# Autodesk Inventor assembly: 13
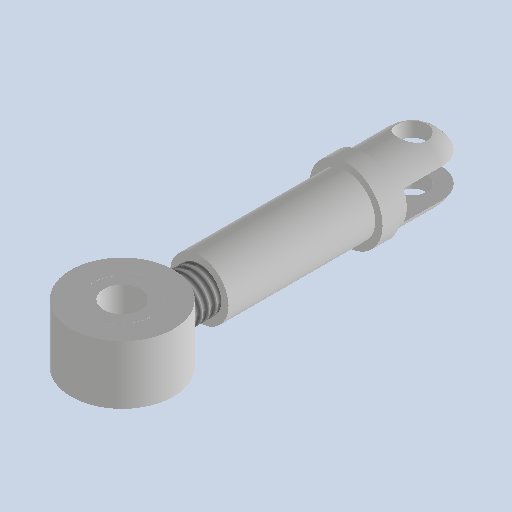
[picture p0: Inventor's stored thumbnail of the model, 512x512]
Saved by Autodesk Inventor 2025.1 (Build 291241000, 241)
## iProperties
Created: 2024-09-13
Part Number: 13
Document SubType Name: Assembly
Designer: ffogue
Author: ffogue
## Documents named in this file (4)
- C:\Users\ffogue\Documents\Inventor\Single cylinder Steam Engine\13.iam
- C:\Users\ffogue\Documents\Inventor\Single cylinder Steam Engine\13 ms.ipt
- C:\Users\ffogue\Documents\Inventor\Single cylinder Steam Engine\13 ms2.ipt
- C:\Users\ffogue\Documents\Inventor\Single cylinder Steam Engine\13.ipt
## Components (3 placed, 3 different names)
1. 13 ms:1 — Mate:1, Flush:1, Mate:2, Rotational:1
2. 13 ms2:1 — Mate:1, Flush:1
3. 13:1 — Mate:2, Rotational:1
## Relationships (4: Mate 2, Flush 1, RevoluteJoint 1)
- Mate:1: 13 ms:1 ↔ 13 ms2:1
- Flush:1: 13 ms:1 ↔ 13 ms2:1
- Mate:2: 13 ms:1 ↔ 13:1
- Rotational:1 [RevoluteJoint]: 13 ms:1 ↔ 13:1
